# Autodesk Inventor assembly: armbox_assembly
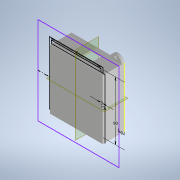
[picture p0: Inventor's stored thumbnail of the model, 180x180]
Saved by Autodesk Inventor 2021 (Build 250183000, 183)
## iProperties
Created: 2021-12-14
Part Number: armbox_assembly
Document SubType Name: Assembly
Designer: marcin
Author: marcin
## Documents named in this file (2)
- C:\Users\marcin\Desktop\Motion_capture\MAIN\Models_3D\Arm_box\armbox_assembly.iam
- C:\Users\marcin\Desktop\Motion_capture\MAIN\Models_3D\Arm_box\arm_box.ipt
## Components (1 placed, 1 different names)
1. arm_box:1 — Mate:1, Mate:2, Mate:3
## Relationships (3: Mate 3)
- Mate:1: arm_box:1
- Mate:2: arm_box:1
- Mate:3: arm_box:1
